# Autodesk Inventor assembly: Bot 1
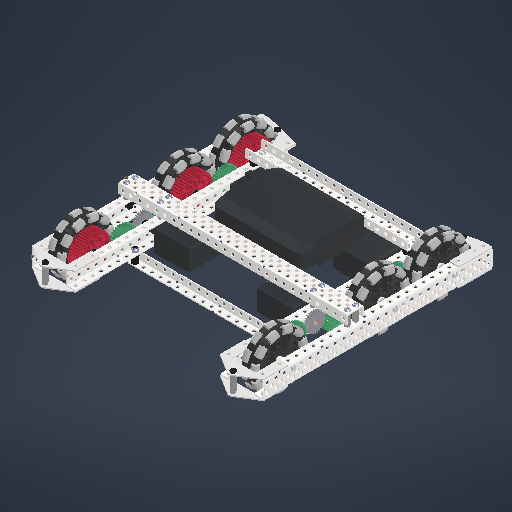
[picture p0: Inventor's stored thumbnail of the model, 512x512]
Saved by Autodesk Inventor 2025.2 (Build 292293000, 293)
## iProperties
Created: 2025-03-17
Part Number: Bot 1
Document SubType Name: Assembly
Designer: Jahan
Author: Jahan
## Documents named in this file (37)
- C:\1629X-7700R-Worlds-Bot\Bot 1\Bot 1.iam
- C:\1629X-7700R-Worlds-Bot\VEX-CAD-Inventor-1.4.2\Structure\C Channel\Aluminum 1x2x1\Alu C 1x2x1x27.ipt
- C:\1629X-7700R-Worlds-Bot\VEX-CAD-Inventor-1.4.2\Structure\C Channel\Aluminum 1x2x1\Alu C 1x2x1x19.ipt
- C:\1629X-7700R-Worlds-Bot\VEX-CAD-Inventor-1.4.2\Motion\Gears\HS Gear.iam
- C:\1629X-7700R-Worlds-Bot\VEX-CAD-Inventor-1.4.2\Motion\Wheels\Omni Wheel\3.25 Omni AS, No Insert.iam
- C:\1629X-7700R-Worlds-Bot\VEX-CAD-Inventor-1.4.2\Motion\Wheels\Omni Wheel.iam
- C:\1629X-7700R-Worlds-Bot\VEX-CAD-Inventor-1.4.2\Motion\Gears\HS Gear\HS 48T Gear, Circle.iam
- C:\1629X-7700R-Worlds-Bot\VEX-CAD-Inventor-1.4.2\Structure\Standoff.ipt
- C:\1629X-7700R-Worlds-Bot\VEX-CAD-Inventor-1.4.2\Structure\Standoff\Standoff .50.ipt
- C:\1629X-7700R-Worlds-Bot\VEX-CAD-Inventor-1.4.2\Motion\Spacers\Washer Teflon.ipt
- C:\1629X-7700R-Worlds-Bot\VEX-CAD-Inventor-1.4.2\Motion\Spacers\Spacer Nylon .375 OD\NSpacer .375 OD x .125.ipt
- C:\1629X-7700R-Worlds-Bot\VEX-CAD-Inventor-1.4.2\Motion\Spacers\Spacer Nylon .375 OD.ipt
- C:\1629X-7700R-Worlds-Bot\VEX-CAD-Inventor-1.4.2\Motion\Spacers\Washer Teflon\TWasher .375 OD x .06250.ipt
- C:\1629X-7700R-Worlds-Bot\VEX-CAD-Inventor-1.4.2\Structure\Hardware\alu_nylock.ipt
- C:\1629X-7700R-Worlds-Bot\VEX-CAD-Inventor-1.4.2\Motion\Gears\LS 36T Gear.ipt
- C:\1629X-7700R-Worlds-Bot\VEX-CAD-Inventor-1.4.2\Motion\Gears\HS Gear\24T HS Gear Cut.iam
- C:\1629X-7700R-Worlds-Bot\VEX-CAD-Inventor-1.4.2\Motion\Shaft LS\Bearing Flat Low Profile.ipt
- C:\1629X-7700R-Worlds-Bot\VEX-CAD-Inventor-1.4.2\Structure\Hardware\Screw Steel - Hex.ipt
- C:\1629X-7700R-Worlds-Bot\VEX-CAD-Inventor-1.4.2\Structure\Hardware\Screw Steel - Hex\SScrew Hex Smooth 1.750.ipt
- C:\1629X-7700R-Worlds-Bot\VEX-CAD-Inventor-1.4.2\Structure\C Channel\Aluminum 1x2x1\Alu C 1x2x1x26.ipt
- C:\1629X-7700R-Worlds-Bot\VEX-CAD-Inventor-1.4.2\Structure\Hardware\Screw Aluminum - Flat Head\AScrew Flat Head Threaded .250.ipt
- C:\1629X-7700R-Worlds-Bot\VEX-CAD-Inventor-1.4.2\Motion\Spacers\Spacer Nylon .375 OD\NSpacer .375 OD x .250.ipt
- C:\1629X-7700R-Worlds-Bot\VEX-CAD-Inventor-1.4.2\Structure\Standoff\Standoff .75.ipt
- C:\1629X-7700R-Worlds-Bot\VEX-CAD-Inventor-1.4.2\Structure\Hardware\Screw Aluminum - Flat Head\AScrew Flat Head Threaded .500.ipt
- C:\1629X-7700R-Worlds-Bot\VEX-CAD-Inventor-1.4.2\Structure\Hardware\Nut Thin Nylock.ipt
- C:\1629X-7700R-Worlds-Bot\VEX-CAD-Inventor-1.4.2\Structure\Hardware\Screw Steel - Star\SScrew Star Smooth .250.ipt
- C:\1629X-7700R-Worlds-Bot\VEX-CAD-Inventor-1.4.2\Structure\Hardware\Screw Steel - Star.ipt
- C:\1629X-7700R-Worlds-Bot\Bot 1\Plastic\backFunnel.ipt
- C:\1629X-7700R-Worlds-Bot\VEX-CAD-Inventor-1.4.2\Structure\Standoff\Standoff 1.00.ipt
- C:\1629X-7700R-Worlds-Bot\VEX-CAD-Inventor-1.4.2\Structure\Angle\Aluminum 1x1\Alu Angle 1x1x19.ipt
- C:\1629X-7700R-Worlds-Bot\VEX-CAD-Inventor-1.4.2\Motion\Spacers\Spacer Nylon .375 OD\NSpacer .375 OD x .500.ipt
- C:\1629X-7700R-Worlds-Bot\VEX-CAD-Inventor-1.4.2\Structure\Hardware\Screw Steel - Star\SScrew Star Smooth .500.ipt
- C:\1629X-7700R-Worlds-Bot\VEX-CAD-Inventor-1.4.2\Electronics\V5 Simple Motor.ipt
- C:\1629X-7700R-Worlds-Bot\VEX-CAD-Inventor-1.4.2\Structure\Hardware\Screw Steel - Star\SScrew Star Smooth .750.ipt
- C:\1629X-7700R-Worlds-Bot\VEX-CAD-Inventor-1.4.2\Structure\Hardware\Screw Nylon - Flat Head\NScrew Flat Head Threaded .250.ipt
- C:\1629X-7700R-Worlds-Bot\VEX-CAD-Inventor-1.4.2\Electronics\V5 Simple Brain.ipt
- C:\1629X-7700R-Worlds-Bot\Bot 1\Plastic\frontFunnel.ipt
## Components (143 placed, 29 different names)
1. Alu C 1x2x1x26:2 — Insert:19, Insert:32, Insert:40, Insert:41, Insert:72, Insert:73, Insert:74, Insert:84, Insert:85, Insert:91, Insert:92, Insert:105, Insert:106, Insert:121, Insert:122, Insert:130, Insert:132, Insert:136, Insert:141, Insert:142, Insert:143, Insert:144, Insert:151, Insert:152, Insert:157, Insert:163, Mate:8, Flush:1, Insert:164, Insert:165, Insert:169
2. Alu C 1x2x1x26:1 — Insert:5, Insert:6, Insert:59, Insert:66, Insert:67, Insert:69, Insert:75, Insert:76, Insert:77, Insert:86, Insert:87, Insert:95, Insert:96, Insert:107, Insert:108, Insert:119, Insert:120, Insert:125, Insert:126, Insert:135, Insert:139, Insert:140, Insert:145, Insert:146, Insert:147, Insert:148, Insert:149, Insert:150, Insert:158
3. Alu C 1x2x1x27:3 — Insert:5, Insert:6, Insert:7, Insert:8, Insert:9, Insert:10
4. Alu C 1x2x1x27:4 — Insert:7, Insert:8, Insert:52, Insert:58, Insert:65, Insert:81, Insert:82, Insert:83, Insert:97, Insert:98, Insert:117, Insert:118, Insert:127, Insert:128, Insert:170, Insert:171, Insert:172, Insert:173
5. Alu C 1x2x1x27:5 — Insert:9, Insert:10, Insert:25, Insert:31, Insert:39, Insert:43, Insert:44, Insert:45, Insert:46, Insert:78, Insert:79, Insert:80, Insert:93, Insert:94, Insert:123, Insert:124, Insert:129, Insert:131, Insert:166, Insert:167, Insert:168
6. LS 36T Gear:1 — Insert:19, Rotation:5, Rotation:6
7. HS 48T Gear, Circle:3 [sub-assembly] — Mate:1, Rotation:4, Rotation:5
8. 3.25 Omni AS, No Insert:4 [sub-assembly] — Mate:1
9. NSpacer .375 OD x .125:2
10. TWasher .375 OD x .06250:2 — Insert:23
11. alu_nylock:3 — Insert:23, Insert:24
12. Standoff .50:3 — Insert:24, Insert:25
13. HS 48T Gear, Circle:4 [sub-assembly] — Mate:2, Rotation:6
14. 3.25 Omni AS, No Insert:5 [sub-assembly] — Mate:2
15. NSpacer .375 OD x .125:3
16. TWasher .375 OD x .06250:3
17. alu_nylock:4
18. Standoff .50:4 — Insert:31
19. LS 36T Gear:2 — Insert:32, Rotation:3, Rotation:4
20. HS 48T Gear, Circle:5 [sub-assembly] — Mate:3, Rotation:1
21. 3.25 Omni AS, No Insert:6 [sub-assembly] — Mate:3
22. NSpacer .375 OD x .125:4
23. TWasher .375 OD x .06250:4
24. alu_nylock:5
25. Standoff .50:5 — Insert:39
26. LS 36T Gear:4 — Insert:40, Rotation:1, Rotation:2
27. NSpacer .375 OD x .125:5 — Insert:41, Insert:71
28. Bearing Flat Low Profile:1 — Insert:43, Insert:44
29. Bearing Flat Low Profile:2 — Insert:45, Insert:46
30. HS 48T Gear, Circle:6 [sub-assembly]
31. 3.25 Omni AS, No Insert:7 [sub-assembly]
32. NSpacer .375 OD x .125:6
33. TWasher .375 OD x .06250:5
34. alu_nylock:6
35. Standoff .50:6 — Insert:52
36. HS 48T Gear, Circle:7 [sub-assembly]
37. 3.25 Omni AS, No Insert:8 [sub-assembly]
38. NSpacer .375 OD x .125:7
39. TWasher .375 OD x .06250:6
40. alu_nylock:7
41. Standoff .50:7 — Insert:58
42. LS 36T Gear:5 — Insert:59
43. HS 48T Gear, Circle:8 [sub-assembly]
44. 3.25 Omni AS, No Insert:9 [sub-assembly]
45. NSpacer .375 OD x .125:8
46. TWasher .375 OD x .06250:7
47. alu_nylock:8
48. Standoff .50:8 — Insert:65
49. LS 36T Gear:6 — Insert:66
50. LS 36T Gear:7 — Insert:67
51. NSpacer .375 OD x .125:9 — Insert:69, Insert:70
52. 24T HS Gear Cut:4 [sub-assembly] — Insert:70
53. 24T HS Gear Cut:5 [sub-assembly] — Insert:71, Rotation:2, Rotation:3
54. SScrew Hex Smooth 1.750:1 — Insert:72
55. SScrew Hex Smooth 1.750:2 — Insert:74
56. SScrew Hex Smooth 1.750:3 — Insert:73
57. SScrew Hex Smooth 1.750:4 — Insert:77
58. SScrew Hex Smooth 1.750:5 — Insert:76
59. SScrew Hex Smooth 1.750:6 — Insert:75
60. AScrew Flat Head Threaded .250:1 — Insert:78
61. AScrew Flat Head Threaded .250:2 — Insert:79
62. AScrew Flat Head Threaded .250:3 — Insert:80
63. AScrew Flat Head Threaded .250:4 — Insert:81
64. AScrew Flat Head Threaded .250:5 — Insert:82
65. AScrew Flat Head Threaded .250:6 — Insert:83
66. Alu C 1x2x1x19:1 — Insert:88, Insert:89, Insert:90, Mate:7, Insert:101, Insert:102, Insert:103, Insert:104
67. NSpacer .375 OD x .250:10 — Insert:84, Insert:88
68. NSpacer .375 OD x .250:11 — Insert:86, Insert:89
69. NSpacer .375 OD x .250:12 — Insert:87, Insert:90
70. NSpacer .375 OD x .250:13 — Insert:85, Mate:7
71. Alu C 1x2x1x27:6 — Insert:99, Insert:100, Insert:109, Insert:110, Insert:111, Insert:112, Insert:113, Insert:114, Insert:115, Insert:116
72. Standoff .75:9 — Insert:94, Insert:99
73. Standoff .75:10 — Insert:91
74. Standoff .75:11 — Insert:92
75. Standoff .75:12 — Insert:98
76. Standoff .75:13 — Insert:97
77. Standoff .75:14 — Insert:95
78. Standoff .75:15 — Insert:93, Insert:100
79. Standoff .75:16 — Insert:96
80. AScrew Flat Head Threaded .500:1 — Insert:101
81. AScrew Flat Head Threaded .500:2 — Insert:104
82. AScrew Flat Head Threaded .500:3 — Insert:102
83. AScrew Flat Head Threaded .500:4 — Insert:103
84. Nut Thin Nylock:1 — Insert:105
85. Nut Thin Nylock:2 — Insert:108
86. Nut Thin Nylock:3 — Insert:106
87. Nut Thin Nylock:4 — Insert:107
88. SScrew Star Smooth .250:1 — Insert:110
89. SScrew Star Smooth .250:2 — Insert:112
90. SScrew Star Smooth .250:3 — Insert:113
91. SScrew Star Smooth .250:4 — Insert:114
92. SScrew Star Smooth .250:5 — Insert:115
93. SScrew Star Smooth .250:6 — Insert:116
94. SScrew Star Smooth .250:7 — Insert:111
95. SScrew Star Smooth .250:8 — Insert:109
96. SScrew Star Smooth .250:9 — Insert:121
97. SScrew Star Smooth .250:10 — Insert:123
98. SScrew Star Smooth .250:11 — Insert:118
99. SScrew Star Smooth .250:12 — Insert:117
100. SScrew Star Smooth .250:13 — Insert:120
101. SScrew Star Smooth .250:14 — Insert:119
102. SScrew Star Smooth .250:15 — Insert:124
103. SScrew Star Smooth .250:16 — Insert:122
104. backFunnel:1 — Insert:125, Insert:127, Insert:159
105. backFunnel:2 — Insert:126, Insert:128, Insert:133, Insert:160
106. backFunnel:3 — Insert:129, Insert:130, Insert:161
107. backFunnel:4 — Insert:131, Insert:132, Insert:134, Insert:162
108. Standoff 1.00:17 — Insert:134
109. Standoff 1.00:18 — Insert:133
110. Alu Angle 1x1x19:1 — Insert:137, Insert:138, Insert:155, Insert:156
111. NSpacer .375 OD x .500:14 — Insert:135, Insert:138
112. NSpacer .375 OD x .500:15 — Insert:136, Insert:137
113. SScrew Star Smooth .500:17 — Insert:141
114. SScrew Star Smooth .500:18 — Insert:146
115. SScrew Star Smooth .500:19 — Insert:144
116. SScrew Star Smooth .500:20 — Insert:145
117. SScrew Star Smooth .500:21 — Insert:143
118. SScrew Star Smooth .500:22 — Insert:139
119. SScrew Star Smooth .500:23 — Insert:140
120. SScrew Star Smooth .500:24 — Insert:142
121. V5 Simple Motor:1 — Insert:147, Insert:148
122. V5 Simple Motor:2 — Insert:149, Insert:150
123. V5 Simple Motor:4 — Insert:151, Insert:152
124. SScrew Star Smooth .750:25 — Insert:156
125. SScrew Star Smooth .750:26 — Insert:155
126. Nut Thin Nylock:5 — Insert:158
127. Nut Thin Nylock:6 — Insert:157
128. NScrew Flat Head Threaded .250:1 — Insert:159
129. NScrew Flat Head Threaded .250:2 — Insert:160
130. NScrew Flat Head Threaded .250:3 — Insert:162
131. NScrew Flat Head Threaded .250:4 — Insert:161
132. V5 Simple Motor:5 — Insert:163, Mate:8
133. V5 Simple Brain:1
134. frontFunnel:1 — Insert:164, Insert:165, Insert:166, Insert:167, Insert:177
135. frontFunnel:2 — Insert:168, Insert:169, Insert:178, Insert:179
136. frontFunnel:3 — Insert:170, Insert:171, Insert:175
137. frontFunnel:4 — Insert:172, Insert:173, Insert:174, Insert:176
138. Standoff 1.00:19 — Insert:179
139. NScrew Flat Head Threaded .250:5 — Insert:177
140. NScrew Flat Head Threaded .250:6 — Insert:178
141. Standoff 1.00:20 — Insert:176
142. NScrew Flat Head Threaded .250:7 — Insert:174
143. NScrew Flat Head Threaded .250:8 — Insert:175
## Relationships (177: Insert 162, Mate 8, RelateRotation 6, Flush 1)
- Insert:5: Alu C 1x2x1x26:1 ↔ Alu C 1x2x1x27:3
- Insert:6: Alu C 1x2x1x26:1 ↔ Alu C 1x2x1x27:3
- Insert:7: Alu C 1x2x1x27:3 ↔ Alu C 1x2x1x27:4
- Insert:8: Alu C 1x2x1x27:3 ↔ Alu C 1x2x1x27:4
- Insert:9: Alu C 1x2x1x27:3 ↔ Alu C 1x2x1x27:5
- Insert:10: Alu C 1x2x1x27:3 ↔ Alu C 1x2x1x27:5
- Insert:19: Alu C 1x2x1x26:2 ↔ LS 36T Gear:1
- [Insert]: HS 48T Gear, Circle:3 ↔ 3.25 Omni AS, No Insert:4
- [Insert]: HS 48T Gear, Circle:3 ↔ NSpacer .375 OD x .125:2
- [Insert]: 3.25 Omni AS, No Insert:4 ↔ TWasher .375 OD x .06250:2
- Insert:23: TWasher .375 OD x .06250:2 ↔ alu_nylock:3
- Insert:24: alu_nylock:3 ↔ Standoff .50:3
- Insert:25: Alu C 1x2x1x27:5 ↔ Standoff .50:3
- [Insert]: HS 48T Gear, Circle:4 ↔ 3.25 Omni AS, No Insert:5
- [Insert]: HS 48T Gear, Circle:4 ↔ NSpacer .375 OD x .125:3
- [Insert]: 3.25 Omni AS, No Insert:5 ↔ TWasher .375 OD x .06250:3
- [Insert]: TWasher .375 OD x .06250:3 ↔ alu_nylock:4
- [Insert]: alu_nylock:4 ↔ Standoff .50:4
- Insert:31: Alu C 1x2x1x27:5 ↔ Standoff .50:4
- Insert:32: Alu C 1x2x1x26:2 ↔ LS 36T Gear:2
- [Insert]: HS 48T Gear, Circle:5 ↔ 3.25 Omni AS, No Insert:6
- [Insert]: HS 48T Gear, Circle:5 ↔ NSpacer .375 OD x .125:4
- [Insert]: 3.25 Omni AS, No Insert:6 ↔ TWasher .375 OD x .06250:4
- [Insert]: TWasher .375 OD x .06250:4 ↔ alu_nylock:5
- [Insert]: alu_nylock:5 ↔ Standoff .50:5
- Insert:39: Alu C 1x2x1x27:5 ↔ Standoff .50:5
- Insert:40: Alu C 1x2x1x26:2 ↔ LS 36T Gear:4
- Mate:1: HS 48T Gear, Circle:3 ↔ 3.25 Omni AS, No Insert:4
- Mate:2: HS 48T Gear, Circle:4 ↔ 3.25 Omni AS, No Insert:5
- Mate:3: HS 48T Gear, Circle:5 ↔ 3.25 Omni AS, No Insert:6
- Insert:41: Alu C 1x2x1x26:2 ↔ NSpacer .375 OD x .125:5
- Insert:43: Alu C 1x2x1x27:5 ↔ Bearing Flat Low Profile:1
- Insert:44: Alu C 1x2x1x27:5 ↔ Bearing Flat Low Profile:1
- Insert:45: Alu C 1x2x1x27:5 ↔ Bearing Flat Low Profile:2
- Insert:46: Alu C 1x2x1x27:5 ↔ Bearing Flat Low Profile:2
- [Insert]: HS 48T Gear, Circle:6 ↔ 3.25 Omni AS, No Insert:7
- [Insert]: HS 48T Gear, Circle:6 ↔ NSpacer .375 OD x .125:6
- [Insert]: 3.25 Omni AS, No Insert:7 ↔ TWasher .375 OD x .06250:5
- [Insert]: TWasher .375 OD x .06250:5 ↔ alu_nylock:6
- [Insert]: alu_nylock:6 ↔ Standoff .50:6
- [Mate]: HS 48T Gear, Circle:6 ↔ 3.25 Omni AS, No Insert:7
- Insert:52: Alu C 1x2x1x27:4 ↔ Standoff .50:6
- [Insert]: HS 48T Gear, Circle:7 ↔ 3.25 Omni AS, No Insert:8
- [Insert]: HS 48T Gear, Circle:7 ↔ NSpacer .375 OD x .125:7
- [Insert]: 3.25 Omni AS, No Insert:8 ↔ TWasher .375 OD x .06250:6
- [Insert]: TWasher .375 OD x .06250:6 ↔ alu_nylock:7
- [Insert]: alu_nylock:7 ↔ Standoff .50:7
- [Mate]: HS 48T Gear, Circle:7 ↔ 3.25 Omni AS, No Insert:8
- Insert:58: Alu C 1x2x1x27:4 ↔ Standoff .50:7
- Insert:59: Alu C 1x2x1x26:1 ↔ LS 36T Gear:5
- [Insert]: HS 48T Gear, Circle:8 ↔ 3.25 Omni AS, No Insert:9
- [Insert]: HS 48T Gear, Circle:8 ↔ NSpacer .375 OD x .125:8
- [Insert]: 3.25 Omni AS, No Insert:9 ↔ TWasher .375 OD x .06250:7
- [Insert]: TWasher .375 OD x .06250:7 ↔ alu_nylock:8
- [Insert]: alu_nylock:8 ↔ Standoff .50:8
- [Mate]: HS 48T Gear, Circle:8 ↔ 3.25 Omni AS, No Insert:9
- Insert:65: Alu C 1x2x1x27:4 ↔ Standoff .50:8
- Insert:66: Alu C 1x2x1x26:1 ↔ LS 36T Gear:6
- Insert:67: Alu C 1x2x1x26:1 ↔ LS 36T Gear:7
- Insert:69: Alu C 1x2x1x26:1 ↔ NSpacer .375 OD x .125:9
- Insert:70: NSpacer .375 OD x .125:9 ↔ 24T HS Gear Cut:4
- Insert:71: NSpacer .375 OD x .125:5 ↔ 24T HS Gear Cut:5
- Insert:72: Alu C 1x2x1x26:2 ↔ SScrew Hex Smooth 1.750:1
- Insert:73: Alu C 1x2x1x26:2 ↔ SScrew Hex Smooth 1.750:3
- Insert:74: Alu C 1x2x1x26:2 ↔ SScrew Hex Smooth 1.750:2
- Insert:75: Alu C 1x2x1x26:1 ↔ SScrew Hex Smooth 1.750:6
- Insert:76: Alu C 1x2x1x26:1 ↔ SScrew Hex Smooth 1.750:5
- Insert:77: Alu C 1x2x1x26:1 ↔ SScrew Hex Smooth 1.750:4
- Insert:78: Alu C 1x2x1x27:5 ↔ AScrew Flat Head Threaded .250:1
- Insert:79: Alu C 1x2x1x27:5 ↔ AScrew Flat Head Threaded .250:2
- Insert:80: Alu C 1x2x1x27:5 ↔ AScrew Flat Head Threaded .250:3
- Insert:81: Alu C 1x2x1x27:4 ↔ AScrew Flat Head Threaded .250:4
- Insert:82: Alu C 1x2x1x27:4 ↔ AScrew Flat Head Threaded .250:5
- Insert:83: Alu C 1x2x1x27:4 ↔ AScrew Flat Head Threaded .250:6
- Insert:84: Alu C 1x2x1x26:2 ↔ NSpacer .375 OD x .250:10
- Insert:85: Alu C 1x2x1x26:2 ↔ NSpacer .375 OD x .250:13
- Insert:86: Alu C 1x2x1x26:1 ↔ NSpacer .375 OD x .250:11
- Insert:87: Alu C 1x2x1x26:1 ↔ NSpacer .375 OD x .250:12
- Insert:88: Alu C 1x2x1x19:1 ↔ NSpacer .375 OD x .250:10
- Insert:89: Alu C 1x2x1x19:1 ↔ NSpacer .375 OD x .250:11
- Insert:90: Alu C 1x2x1x19:1 ↔ NSpacer .375 OD x .250:12
- Mate:7: Alu C 1x2x1x19:1 ↔ NSpacer .375 OD x .250:13
- Insert:91: Alu C 1x2x1x26:2 ↔ Standoff .75:10
- Insert:92: Alu C 1x2x1x26:2 ↔ Standoff .75:11
- Insert:93: Alu C 1x2x1x27:5 ↔ Standoff .75:15
- Insert:94: Alu C 1x2x1x27:5 ↔ Standoff .75:9
- Insert:95: Alu C 1x2x1x26:1 ↔ Standoff .75:14
- Insert:96: Alu C 1x2x1x26:1 ↔ Standoff .75:16
- Insert:97: Alu C 1x2x1x27:4 ↔ Standoff .75:13
- Insert:98: Alu C 1x2x1x27:4 ↔ Standoff .75:12
- Insert:99: Alu C 1x2x1x27:6 ↔ Standoff .75:9
- Insert:100: Alu C 1x2x1x27:6 ↔ Standoff .75:15
- Insert:101: Alu C 1x2x1x19:1 ↔ AScrew Flat Head Threaded .500:1
- Insert:102: Alu C 1x2x1x19:1 ↔ AScrew Flat Head Threaded .500:3
- Insert:103: Alu C 1x2x1x19:1 ↔ AScrew Flat Head Threaded .500:4
- Insert:104: Alu C 1x2x1x19:1 ↔ AScrew Flat Head Threaded .500:2
- Insert:105: Alu C 1x2x1x26:2 ↔ Nut Thin Nylock:1
- Insert:106: Alu C 1x2x1x26:2 ↔ Nut Thin Nylock:3
- Insert:107: Alu C 1x2x1x26:1 ↔ Nut Thin Nylock:4
- Insert:108: Alu C 1x2x1x26:1 ↔ Nut Thin Nylock:2
- Insert:109: Alu C 1x2x1x27:6 ↔ SScrew Star Smooth .250:8
- Insert:110: Alu C 1x2x1x27:6 ↔ SScrew Star Smooth .250:1
- Insert:111: Alu C 1x2x1x27:6 ↔ SScrew Star Smooth .250:7
- Insert:112: Alu C 1x2x1x27:6 ↔ SScrew Star Smooth .250:2
- Insert:113: Alu C 1x2x1x27:6 ↔ SScrew Star Smooth .250:3
- Insert:114: Alu C 1x2x1x27:6 ↔ SScrew Star Smooth .250:4
- Insert:115: Alu C 1x2x1x27:6 ↔ SScrew Star Smooth .250:5
- Insert:116: Alu C 1x2x1x27:6 ↔ SScrew Star Smooth .250:6
- Insert:117: Alu C 1x2x1x27:4 ↔ SScrew Star Smooth .250:12
- Insert:118: Alu C 1x2x1x27:4 ↔ SScrew Star Smooth .250:11
- Insert:119: Alu C 1x2x1x26:1 ↔ SScrew Star Smooth .250:14
- Insert:120: Alu C 1x2x1x26:1 ↔ SScrew Star Smooth .250:13
- Insert:121: Alu C 1x2x1x26:2 ↔ SScrew Star Smooth .250:9
- Insert:122: Alu C 1x2x1x26:2 ↔ SScrew Star Smooth .250:16
- Insert:123: Alu C 1x2x1x27:5 ↔ SScrew Star Smooth .250:10
- Insert:124: Alu C 1x2x1x27:5 ↔ SScrew Star Smooth .250:15
- Insert:125: Alu C 1x2x1x26:1 ↔ backFunnel:1
- Insert:126: Alu C 1x2x1x26:1 ↔ backFunnel:2
- Insert:127: Alu C 1x2x1x27:4 ↔ backFunnel:1
- Insert:128: Alu C 1x2x1x27:4 ↔ backFunnel:2
- Insert:129: Alu C 1x2x1x27:5 ↔ backFunnel:3
- Insert:130: Alu C 1x2x1x26:2 ↔ backFunnel:3
- Insert:131: Alu C 1x2x1x27:5 ↔ backFunnel:4
- Insert:132: Alu C 1x2x1x26:2 ↔ backFunnel:4
- Insert:133: backFunnel:2 ↔ Standoff 1.00:18
- Insert:134: backFunnel:4 ↔ Standoff 1.00:17
- Insert:135: Alu C 1x2x1x26:1 ↔ NSpacer .375 OD x .500:14
- Insert:136: Alu C 1x2x1x26:2 ↔ NSpacer .375 OD x .500:15
- Insert:137: Alu Angle 1x1x19:1 ↔ NSpacer .375 OD x .500:15
- Insert:138: Alu Angle 1x1x19:1 ↔ NSpacer .375 OD x .500:14
- Insert:139: Alu C 1x2x1x26:1 ↔ SScrew Star Smooth .500:22
- Insert:140: Alu C 1x2x1x26:1 ↔ SScrew Star Smooth .500:23
- Insert:141: Alu C 1x2x1x26:2 ↔ SScrew Star Smooth .500:17
- Insert:142: Alu C 1x2x1x26:2 ↔ SScrew Star Smooth .500:24
- Insert:143: Alu C 1x2x1x26:2 ↔ SScrew Star Smooth .500:21
- Insert:144: Alu C 1x2x1x26:2 ↔ SScrew Star Smooth .500:19
- Insert:145: Alu C 1x2x1x26:1 ↔ SScrew Star Smooth .500:20
- Insert:146: Alu C 1x2x1x26:1 ↔ SScrew Star Smooth .500:18
- Insert:147: Alu C 1x2x1x26:1 ↔ V5 Simple Motor:1
- Insert:148: Alu C 1x2x1x26:1 ↔ V5 Simple Motor:1
- Insert:149: Alu C 1x2x1x26:1 ↔ V5 Simple Motor:2
- Insert:150: Alu C 1x2x1x26:1 ↔ V5 Simple Motor:2
- Insert:151: Alu C 1x2x1x26:2 ↔ V5 Simple Motor:4
- Insert:152: Alu C 1x2x1x26:2 ↔ V5 Simple Motor:4
- Insert:155: Alu Angle 1x1x19:1 ↔ SScrew Star Smooth .750:26
- Insert:156: Alu Angle 1x1x19:1 ↔ SScrew Star Smooth .750:25
- Insert:157: Alu C 1x2x1x26:2 ↔ Nut Thin Nylock:6
- Insert:158: Alu C 1x2x1x26:1 ↔ Nut Thin Nylock:5
- Insert:159: backFunnel:1 ↔ NScrew Flat Head Threaded .250:1
- Insert:160: backFunnel:2 ↔ NScrew Flat Head Threaded .250:2
- Insert:161: backFunnel:3 ↔ NScrew Flat Head Threaded .250:4
- Insert:162: backFunnel:4 ↔ NScrew Flat Head Threaded .250:3
- Insert:163: Alu C 1x2x1x26:2 ↔ V5 Simple Motor:5
- Mate:8: Alu C 1x2x1x26:2 ↔ V5 Simple Motor:5
- Flush:1: Alu C 1x2x1x26:2
- Insert:164: Alu C 1x2x1x26:2 ↔ frontFunnel:1
- Insert:165: Alu C 1x2x1x26:2 ↔ frontFunnel:1
- Insert:166: Alu C 1x2x1x27:5 ↔ frontFunnel:1
- Insert:167: Alu C 1x2x1x27:5 ↔ frontFunnel:1
- Insert:168: Alu C 1x2x1x27:5 ↔ frontFunnel:2
- Insert:169: Alu C 1x2x1x26:2 ↔ frontFunnel:2
- Insert:170: Alu C 1x2x1x27:4 ↔ frontFunnel:3
- Insert:171: Alu C 1x2x1x27:4 ↔ frontFunnel:3
- Insert:172: Alu C 1x2x1x27:4 ↔ frontFunnel:4
- Insert:173: Alu C 1x2x1x27:4 ↔ frontFunnel:4
- Insert:174: frontFunnel:4 ↔ NScrew Flat Head Threaded .250:7
- Insert:175: frontFunnel:3 ↔ NScrew Flat Head Threaded .250:8
- Insert:176: frontFunnel:4 ↔ Standoff 1.00:20
- Insert:177: frontFunnel:1 ↔ NScrew Flat Head Threaded .250:5
- Insert:178: frontFunnel:2 ↔ NScrew Flat Head Threaded .250:6
- Insert:179: frontFunnel:2 ↔ Standoff 1.00:19
- Rotation:1 [RelateRotation] (1.3333 ul): HS 48T Gear, Circle:5 ↔ LS 36T Gear:4
- Rotation:2 [RelateRotation] (1.5 ul): LS 36T Gear:4 ↔ 24T HS Gear Cut:5
- Rotation:3 [RelateRotation] (0.6667 ul): LS 36T Gear:2 ↔ 24T HS Gear Cut:5
- Rotation:4 [RelateRotation] (0.75 ul): HS 48T Gear, Circle:3 ↔ LS 36T Gear:2
- Rotation:5 [RelateRotation] (1.3333 ul): LS 36T Gear:1 ↔ HS 48T Gear, Circle:3
- Rotation:6 [RelateRotation] (0.75 ul): LS 36T Gear:1 ↔ HS 48T Gear, Circle:4
## Named parameters: d122_d116 = 0 mm, d123_d117 = 0 mm, d124_d119 = 0 mm, d129_d122_d116 = 0 mm, d130_d123_d117 = 0 mm, d131_d124_d119 = 0 mm, d132_d126 = 0 mm, d133_d127 = 0 mm, d144_d129_d122_d116 = 0 mm, d145_d130_d123_d117 = 0 mm, d146_d131_d124_d119 = 0 mm, d147_d132_d126 = 0 mm, d148_d133_d127 = 0 mm, d162_d127 = 0 mm, d163_d153 = 0 mm, d164_d122_d116 = 0 mm, d165_d123_d117 = 0 mm, d166_d124_d119 = 0 mm, d167_d126 = 0 mm, d169_d127 = 0 mm, d170_d153 = 0 mm, d171_d122_d116 = 0 mm, d172_d123_d117 = 0 mm, d173_d124_d119 = 0 mm, d174_d126 = 0 mm, d177_d169_d127 = 0 mm, d178_d170_d153 = 0 mm, d179_d171_d122_d116 = 0 mm, d180_d172_d123_d117 = 0 mm, d181_d173_d124_d119 = 0 mm, d182_d174_d126 = 0 mm
